# Autodesk Inventor assembly: Bucket Assm
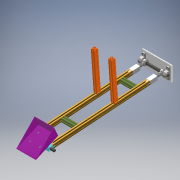
[picture p0: Inventor's stored thumbnail of the model, 180x180]
Saved by Autodesk Inventor 2020 (Build 240168000, 168)
## iProperties
Created: 2019-10-01
Part Number: Bucket Assm
Document SubType Name: Assembly
Designer: Matt
Author: Matt
## Documents named in this file (11)
- C:\Users\Matt\OneDrive\Inventor\NASA 2020\NASA 20\NASA-20\NASA-20\Bucket Assm.iam
- C:\Users\Matt\OneDrive\Inventor\NASA 2020\NASA 20\NASA-20\NASA-20\Matt Bucket\Arm Support Plate.ipt
- C:\Users\Matt\OneDrive\Inventor\NASA 2020\NASA 20\NASA-20\NASA-20\Matt Bucket\5912K400_OIL-EMBEDDED MOUNTED SLEEVE BEARING.ipt
- C:\Users\Matt\OneDrive\Inventor\NASA 2020\NASA 20\NASA-20\NASA-20\Matt Bucket\Arm Pivot.ipt
- C:\Users\Matt\OneDrive\Inventor\NASA 2020\NASA 20\NASA-20\NASA-20\Matt Bucket\3798K490_FULLY THREADED C1035 STEEL ROD END.ipt
- C:\Users\Matt\OneDrive\Inventor\NASA 2020\NASA 20\NASA-20\NASA-20\Matt Bucket\Line 5 Adapter.ipt
- C:\Users\Matt\OneDrive\Inventor\NASA 2020\NASA 20\NASA-20\NASA-20\Matt Bucket\Arm Line5.ipt
- C:\Users\Matt\OneDrive\Inventor\NASA 2020\NASA 20\NASA-20\NASA-20\Matt Bucket\Line5 A Frame Legs.ipt
- C:\Users\Matt\OneDrive\Inventor\NASA 2020\NASA 20\NASA-20\NASA-20\Matt Bucket\Line 5 Bucket Adapter.ipt
- C:\Users\Matt\OneDrive\Inventor\NASA 2020\NASA 20\NASA-20\NASA-20\Matt Bucket\Bucket.ipt
- C:\Users\Matt\OneDrive\Inventor\NASA 2020\NASA 20\NASA-20\NASA-20\Matt Bucket\Line 5 Arm Braces.ipt
## Components (20 placed, 10 different names)
1. Arm Support Plate:1 — Rotational:1, Mate:1, Rotational:2, Mate:2, Flush:1
2. 5912K400_OIL-EMBEDDED MOUNTED SLEEVE BEARING:1 — Rotational:1, Mate:1, Mate:18
3. 5912K400_OIL-EMBEDDED MOUNTED SLEEVE BEARING:2 — Rotational:2, Mate:2, Mate:3
4. Arm Pivot:1 — Mate:3, Flush:1, Mate:4, Mate:17, Flush:15
5. 3798K490_FULLY THREADED C1035 STEEL ROD END:1 — Flush:2, Mate:9, Mate:17, Mate:18
6. 3798K490_FULLY THREADED C1035 STEEL ROD END:2 — Mate:4, Flush:2, Mate:10, Mate:11
7. Line 5 Adapter:1 — Mate:10, Flush:3, Mate:11, Flush:4, Mate:13, Mate:14, Flush:6, Flush:10
8. Line 5 Adapter:2 — Mate:9, Flush:3, Flush:4, Mate:12, Mate:15, Flush:5
9. Arm Line5:1 — Mate:13, Mate:14, Flush:6, Mate:16, Mate:20, Flush:8, Mate:22, Flush:11, Flush:14, Mate:33, Flush:16
10. Arm Line5:2 — Mate:12, Mate:15, Flush:5, Mate:16, Mate:19, Flush:7, Mate:21, Flush:12, Flush:13, Mate:34, Flush:17
11. Line5 A Frame Legs:1 — Mate:19, Flush:7, Flush:9
12. Line5 A Frame Legs:2 — Mate:20, Flush:8, Flush:9, Flush:10
13. Line 5 Bucket Adapter:1 — Mate:22, Flush:11, Flush:14, Mate:23, Angle:1
14. Line 5 Bucket Adapter:2 — Mate:21, Flush:12, Flush:13, Mate:32
15. Arm Pivot:2 — Mate:23, Flush:15, Mate:26, Mate:27
16. Bucket:1 — Mate:24, Mate:25, Mate:28, Mate:29, Mate:30, Mate:31, Angle:1
17. 5912K400_OIL-EMBEDDED MOUNTED SLEEVE BEARING:3 — Mate:25, Mate:27, Mate:28, Mate:29, Mate:32
18. 5912K400_OIL-EMBEDDED MOUNTED SLEEVE BEARING:4 — Mate:24, Mate:26, Mate:30, Mate:31
19. Line 5 Arm Braces:1 — Mate:33, Flush:16
20. Line 5 Arm Braces:2 — Mate:34, Flush:17
## Relationships (50: Mate 30, Flush 17, RevoluteJoint 2, Angle 1)
- Rotational:1 [RevoluteJoint]: Arm Support Plate:1 ↔ 5912K400_OIL-EMBEDDED MOUNTED SLEEVE BEARING:1
- Mate:1: Arm Support Plate:1 ↔ 5912K400_OIL-EMBEDDED MOUNTED SLEEVE BEARING:1
- Rotational:2 [RevoluteJoint]: Arm Support Plate:1 ↔ 5912K400_OIL-EMBEDDED MOUNTED SLEEVE BEARING:2
- Mate:2: Arm Support Plate:1 ↔ 5912K400_OIL-EMBEDDED MOUNTED SLEEVE BEARING:2
- Mate:3: 5912K400_OIL-EMBEDDED MOUNTED SLEEVE BEARING:2 ↔ Arm Pivot:1
- Flush:1: Arm Support Plate:1 ↔ Arm Pivot:1
- Mate:4: Arm Pivot:1 ↔ 3798K490_FULLY THREADED C1035 STEEL ROD END:2
- Flush:2: 3798K490_FULLY THREADED C1035 STEEL ROD END:1 ↔ 3798K490_FULLY THREADED C1035 STEEL ROD END:2
- Mate:9: 3798K490_FULLY THREADED C1035 STEEL ROD END:1 ↔ Line 5 Adapter:2
- Mate:10: 3798K490_FULLY THREADED C1035 STEEL ROD END:2 ↔ Line 5 Adapter:1
- Flush:3: Line 5 Adapter:1 ↔ Line 5 Adapter:2
- Mate:11: 3798K490_FULLY THREADED C1035 STEEL ROD END:2 ↔ Line 5 Adapter:1
- Flush:4: Line 5 Adapter:1 ↔ Line 5 Adapter:2
- Mate:12: Line 5 Adapter:2 ↔ Arm Line5:2
- Mate:13: Line 5 Adapter:1 ↔ Arm Line5:1
- Mate:14: Line 5 Adapter:1 ↔ Arm Line5:1
- Mate:15: Line 5 Adapter:2 ↔ Arm Line5:2
- Flush:5: Line 5 Adapter:2 ↔ Arm Line5:2
- Flush:6: Line 5 Adapter:1 ↔ Arm Line5:1
- Mate:16 (69.85 mm): Arm Line5:1 ↔ Arm Line5:2
- Mate:17: Arm Pivot:1 ↔ 3798K490_FULLY THREADED C1035 STEEL ROD END:1
- Mate:18 (4.2926 mm): 5912K400_OIL-EMBEDDED MOUNTED SLEEVE BEARING:1 ↔ 3798K490_FULLY THREADED C1035 STEEL ROD END:1
- Mate:19: Arm Line5:2 ↔ Line5 A Frame Legs:1
- Mate:20: Arm Line5:1 ↔ Line5 A Frame Legs:2
- Flush:7: Arm Line5:2 ↔ Line5 A Frame Legs:1
- Flush:8: Arm Line5:1 ↔ Line5 A Frame Legs:2
- Flush:9: Line5 A Frame Legs:1 ↔ Line5 A Frame Legs:2
- Flush:10 (203.2 mm): Line 5 Adapter:1 ↔ Line5 A Frame Legs:2
- Mate:21: Arm Line5:2 ↔ Line 5 Bucket Adapter:2
- Mate:22: Arm Line5:1 ↔ Line 5 Bucket Adapter:1
- Flush:11: Arm Line5:1 ↔ Line 5 Bucket Adapter:1
- Flush:12: Arm Line5:2 ↔ Line 5 Bucket Adapter:2
- Flush:13: Arm Line5:2 ↔ Line 5 Bucket Adapter:2
- Flush:14: Arm Line5:1 ↔ Line 5 Bucket Adapter:1
- Mate:23: Line 5 Bucket Adapter:1 ↔ Arm Pivot:2
- Flush:15: Arm Pivot:1 ↔ Arm Pivot:2
- Mate:24: Bucket:1 ↔ 5912K400_OIL-EMBEDDED MOUNTED SLEEVE BEARING:4
- Mate:25: Bucket:1 ↔ 5912K400_OIL-EMBEDDED MOUNTED SLEEVE BEARING:3
- Mate:26: Arm Pivot:2 ↔ 5912K400_OIL-EMBEDDED MOUNTED SLEEVE BEARING:4
- Mate:27: Arm Pivot:2 ↔ 5912K400_OIL-EMBEDDED MOUNTED SLEEVE BEARING:3
- Mate:28: Bucket:1 ↔ 5912K400_OIL-EMBEDDED MOUNTED SLEEVE BEARING:3
- Mate:29: Bucket:1 ↔ 5912K400_OIL-EMBEDDED MOUNTED SLEEVE BEARING:3
- Mate:30: Bucket:1 ↔ 5912K400_OIL-EMBEDDED MOUNTED SLEEVE BEARING:4
- Mate:31: Bucket:1 ↔ 5912K400_OIL-EMBEDDED MOUNTED SLEEVE BEARING:4
- Mate:32 (1.5875 mm): Line 5 Bucket Adapter:2 ↔ 5912K400_OIL-EMBEDDED MOUNTED SLEEVE BEARING:3
- Mate:33: Arm Line5:1 ↔ Line 5 Arm Braces:1
- Flush:16: Arm Line5:1 ↔ Line 5 Arm Braces:1
- Mate:34: Arm Line5:2 ↔ Line 5 Arm Braces:2
- Flush:17: Arm Line5:2 ↔ Line 5 Arm Braces:2
- Angle:1 (110 deg): Line 5 Bucket Adapter:1 ↔ Bucket:1
